# Autodesk Inventor assembly: 000 Ensamblaje 3d_LM-Cable_Forming - BOT00
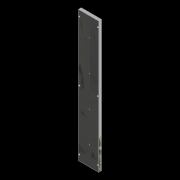
[picture p0: Inventor's stored thumbnail of the model, 180x180]
Saved by Autodesk Inventor 2018.3 (Build 223284000, 284)
## iProperties
Created: 2026-02-12
Part Number: 000 Ensamblaje 3d_LM-Cable_Forming - BOT00
Document SubType Name: Assembly
Designer: aca6
Manufacturer-1: {"Name": "Embention Sistemas Inteligentes S.A.", "PartNumber": "3d_LM-Cable_Forming - BOT00", "Link": ""}
Manufacturer-2: {"Name": "", "PartNumber": "", "Link": ""}
Manufacturer-3: {"Name": "", "PartNumber": "", "Link": ""}
Manufacturer-4: {"Name": "", "PartNumber": "", "Link": ""}
Manufacturer-5: {"Name": "", "PartNumber": "", "Link": ""}
Provider-1: {"Name": "", "PartNumber": "", "Link": ""}
Provider-2: {"Name": "", "PartNumber": "", "Link": ""}
Provider-3: {"Name": "", "PartNumber": "", "Link": ""}
Provider-4: {"Name": "", "PartNumber": "", "Link": ""}
Provider-5: {"Name": "", "PartNumber": "", "Link": ""}
Author: aca6
## Documents named in this file (4)
- C:\Users\aca6\git\LM\items\3d_LM\items\LM-Cable_Forming\3d_LM-Cable_Forming\variants\BOT00\variants\000 Ensamblaje 3d_LM-Cable_Forming - BOT00.iam
- C:\Users\aca6\git\LM\items\3d_LM\items\LM-Cable_Forming\3d_LM-Cable_Forming\variants\BOT00\3d\3d_LM-Cable_Forming - Bot mold.ipt
- C:\Users\aca6\git\LM\items\3d_LM\3d\3d_LM - Bottom Wire - Phantom.ipt
- C:\Users\aca6\git\LM\items\_accesories\Pasadores\3d_Fabory\3d\DIN 7\DIN 7 4x8 mm Inox A4.ipt
## Components (9 placed, 3 different names)
1. 3d_LM-Cable_Forming - Bot mold:1 — Mate:1, Flush:1, Flush:2, Mate:2, Mate:3, Flush:4, Mate:9, Flush:5, Flush:6, Flush:7, Flush:8, Flush:9
2. 3d_LM-Cable_Forming - Bot mold:2 — Mate:1, Flush:1, Flush:2, Flush:3, Mate:4, Mate:5, Mate:6, Mate:7, Mate:8
3. 3d_LM - Bottom Wire - Phantom:1 — Flush:3, Mate:2, Mate:3
4. DIN 7 4x8 mm Inox A4:1 — Mate:4, Flush:4
5. DIN 7 4x8 mm Inox A4:2 — Mate:9, Flush:5
6. DIN 7 4x8 mm Inox A4:3 — Mate:6, Flush:6
7. DIN 7 4x8 mm Inox A4:4 — Mate:5, Flush:7
8. DIN 7 4x8 mm Inox A4:5 — Mate:8, Flush:8
9. DIN 7 4x8 mm Inox A4:6 — Mate:7, Flush:9
## Relationships (18: Mate 9, Flush 9)
- Mate:1: 3d_LM-Cable_Forming - Bot mold:1 ↔ 3d_LM-Cable_Forming - Bot mold:2
- Flush:1: 3d_LM-Cable_Forming - Bot mold:1 ↔ 3d_LM-Cable_Forming - Bot mold:2
- Flush:2: 3d_LM-Cable_Forming - Bot mold:1 ↔ 3d_LM-Cable_Forming - Bot mold:2
- Flush:3: 3d_LM-Cable_Forming - Bot mold:2 ↔ 3d_LM - Bottom Wire - Phantom:1
- Mate:2: 3d_LM-Cable_Forming - Bot mold:1 ↔ 3d_LM - Bottom Wire - Phantom:1
- Mate:3: 3d_LM-Cable_Forming - Bot mold:1 ↔ 3d_LM - Bottom Wire - Phantom:1
- Mate:4: 3d_LM-Cable_Forming - Bot mold:2 ↔ DIN 7 4x8 mm Inox A4:1
- Mate:5: 3d_LM-Cable_Forming - Bot mold:2 ↔ DIN 7 4x8 mm Inox A4:4
- Mate:6: 3d_LM-Cable_Forming - Bot mold:2 ↔ DIN 7 4x8 mm Inox A4:3
- Mate:7: 3d_LM-Cable_Forming - Bot mold:2 ↔ DIN 7 4x8 mm Inox A4:6
- Mate:8: 3d_LM-Cable_Forming - Bot mold:2 ↔ DIN 7 4x8 mm Inox A4:5
- Flush:4: 3d_LM-Cable_Forming - Bot mold:1 ↔ DIN 7 4x8 mm Inox A4:1
- Mate:9: 3d_LM-Cable_Forming - Bot mold:1 ↔ DIN 7 4x8 mm Inox A4:2
- Flush:5: 3d_LM-Cable_Forming - Bot mold:1 ↔ DIN 7 4x8 mm Inox A4:2
- Flush:6: 3d_LM-Cable_Forming - Bot mold:1 ↔ DIN 7 4x8 mm Inox A4:3
- Flush:7: 3d_LM-Cable_Forming - Bot mold:1 ↔ DIN 7 4x8 mm Inox A4:4
- Flush:8: 3d_LM-Cable_Forming - Bot mold:1 ↔ DIN 7 4x8 mm Inox A4:5
- Flush:9: 3d_LM-Cable_Forming - Bot mold:1 ↔ DIN 7 4x8 mm Inox A4:6
